# Autodesk Inventor assembly: HipRight
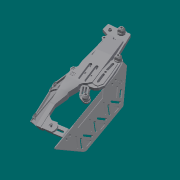
[picture p0: Inventor's stored thumbnail of the model, 180x180]
Saved by Autodesk Inventor 2015 SP1 (Build 190203100, 203)
## iProperties
Created: 2014-09-01
Part Number: HipRight
Document SubType Name: Assembly
Designer: Inventor
Mass: 809.946 g
Surface Area: 1272.46 cm^2
Volume: 359.464 cm^3
Density: 2.2532 g/cm^3
Author: Inventor
## Documents named in this file (7)
- C:\Users\Val\Desktop\ExoGit\elysium-max-exoskeleton\src\Assemblies\HipRight.iam
- C:\Users\Val\Desktop\ExoGit\elysium-max-exoskeleton\src\SpacerShort.ipt
- C:\Users\Val\Desktop\ExoGit\elysium-max-exoskeleton\src\HipRight.ipt
- C:\Users\Val\Desktop\ExoGit\elysium-max-exoskeleton\src\HipTopConnectorRight.ipt
- C:\Users\Val\Desktop\ExoGit\elysium-max-exoskeleton\src\HipBottomConnectorRight.ipt
- C:\Users\Val\Desktop\ExoGit\elysium-max-exoskeleton\src\HipShockPlateRight.ipt
- C:\Users\Val\Desktop\ExoGit\elysium-max-exoskeleton\src\HipPistonConnectorRight.ipt
## Components (8 placed, 6 different names)
1. HipRight:1 — Mate:24, Mate:25, Mate:26, Angle:4, Angle:5, Mate:27, Mate:28, Mate:31, Mate:32, Mate:33, Mate:34, Mate:35, Mate:36
2. HipTopConnectorRight:1 — Mate:24, Mate:25, Mate:26, Angle:4, Mate:30, Angle:6
3. HipBottomConnectorRight:1 — Angle:5, Mate:27, Mate:28, Mate:29
4. HipShockPlateRight:1 — Mate:29, Mate:30, Angle:6
5. HipPistonConnectorRight:1 — Mate:31, Mate:32, Mate:37, Mate:38
6. SpacerShort:4 — Mate:33, Mate:34
7. SpacerShort:5 — Mate:35, Mate:36
8. SpacerShort:6 — Mate:37, Mate:38
## Relationships (18: Mate 15, Angle 3)
- Mate:24: HipRight:1 ↔ HipTopConnectorRight:1
- Mate:25: HipRight:1 ↔ HipTopConnectorRight:1
- Mate:26: HipRight:1 ↔ HipTopConnectorRight:1
- Angle:4 (180 deg): HipRight:1 ↔ HipTopConnectorRight:1
- Angle:5 (0 deg): HipRight:1 ↔ HipBottomConnectorRight:1
- Mate:27: HipRight:1 ↔ HipBottomConnectorRight:1
- Mate:28: HipRight:1 ↔ HipBottomConnectorRight:1
- Mate:29: HipBottomConnectorRight:1 ↔ HipShockPlateRight:1
- Mate:30: HipTopConnectorRight:1 ↔ HipShockPlateRight:1
- Angle:6 (180 deg): HipTopConnectorRight:1 ↔ HipShockPlateRight:1
- Mate:31: HipRight:1 ↔ HipPistonConnectorRight:1
- Mate:32: HipRight:1 ↔ HipPistonConnectorRight:1
- Mate:33: HipRight:1 ↔ SpacerShort:4
- Mate:34: HipRight:1 ↔ SpacerShort:4
- Mate:35: HipRight:1 ↔ SpacerShort:5
- Mate:36: HipRight:1 ↔ SpacerShort:5
- Mate:37: HipPistonConnectorRight:1 ↔ SpacerShort:6
- Mate:38: HipPistonConnectorRight:1 ↔ SpacerShort:6
